# Autodesk Inventor assembly: 0008-10-02 X Axis
(part 2 of 2)
- [Insert] (2 mm): 0008-10-2018 DIN 912 - M4 x 0.7 x 40.ipt:220 ↔ 0008-10-2001 DIN 934 - M4 x 0.7.ipt:222
- [Insert]: 0008-10-2002 DIN 125 - A 4.3.ipt:225 ↔ 0008-10-2001 DIN 934 - M4 x 0.7.ipt:226
- [Insert]: 0008-10-2018 DIN 912 - M4 x 0.7 x 40.ipt:224 ↔ 0008-10-2002 DIN 125 - A 4.3.ipt:227
- [Insert] (2 mm): 0008-10-2018 DIN 912 - M4 x 0.7 x 40.ipt:224 ↔ 0008-10-2001 DIN 934 - M4 x 0.7.ipt:226
- Insert:124: 0008-10-008 X Axis suport.ipt:10 ↔ 0008-10-2002 DIN 125 - A 4.3.ipt:219
- Insert:125: 0008-10-008 X Axis suport.ipt:10 ↔ 0008-10-2002 DIN 125 - A 4.3.ipt:223
- Insert:126: 0008-10-008 X Axis suport.ipt:10 ↔ 0008-10-2002 DIN 125 - A 4.3.ipt:215
- Insert:127: 0008-10-008 X Axis suport.ipt:10 ↔ 0008-10-2002 DIN 125 - A 4.3.ipt:227
- [Insert]: 0008-10-2002 DIN 125 - A 4.3.ipt:229 ↔ 0008-10-2001 DIN 934 - M4 x 0.7.ipt:230
- [Insert]: 0008-10-2018 DIN 912 - M4 x 0.7 x 40.ipt:228 ↔ 0008-10-2002 DIN 125 - A 4.3.ipt:231
- [Insert] (2 mm): 0008-10-2018 DIN 912 - M4 x 0.7 x 40.ipt:228 ↔ 0008-10-2001 DIN 934 - M4 x 0.7.ipt:230
- [Insert]: 0008-10-2002 DIN 125 - A 4.3.ipt:233 ↔ 0008-10-2001 DIN 934 - M4 x 0.7.ipt:234
- [Insert]: 0008-10-2018 DIN 912 - M4 x 0.7 x 40.ipt:232 ↔ 0008-10-2002 DIN 125 - A 4.3.ipt:235
- [Insert] (2 mm): 0008-10-2018 DIN 912 - M4 x 0.7 x 40.ipt:232 ↔ 0008-10-2001 DIN 934 - M4 x 0.7.ipt:234
- [Insert]: 0008-10-2002 DIN 125 - A 4.3.ipt:237 ↔ 0008-10-2001 DIN 934 - M4 x 0.7.ipt:238
- [Insert]: 0008-10-2018 DIN 912 - M4 x 0.7 x 40.ipt:236 ↔ 0008-10-2002 DIN 125 - A 4.3.ipt:239
- [Insert] (2 mm): 0008-10-2018 DIN 912 - M4 x 0.7 x 40.ipt:236 ↔ 0008-10-2001 DIN 934 - M4 x 0.7.ipt:238
- [Insert]: 0008-10-2002 DIN 125 - A 4.3.ipt:241 ↔ 0008-10-2001 DIN 934 - M4 x 0.7.ipt:242
- [Insert]: 0008-10-2018 DIN 912 - M4 x 0.7 x 40.ipt:240 ↔ 0008-10-2002 DIN 125 - A 4.3.ipt:243
- [Insert] (2 mm): 0008-10-2018 DIN 912 - M4 x 0.7 x 40.ipt:240 ↔ 0008-10-2001 DIN 934 - M4 x 0.7.ipt:242
- Insert:140: 0008-10-009 X Axis suport.ipt:9 ↔ 0008-10-2002 DIN 125 - A 4.3.ipt:243
- Insert:141: 0008-10-009 X Axis suport.ipt:9 ↔ 0008-10-2002 DIN 125 - A 4.3.ipt:231
- Insert:142: 0008-10-009 X Axis suport.ipt:9 ↔ 0008-10-2002 DIN 125 - A 4.3.ipt:235
- Insert:143: 0008-10-009 X Axis suport.ipt:9 ↔ 0008-10-2002 DIN 125 - A 4.3.ipt:239
- [Insert]: 0008-10-2002 DIN 125 - A 4.3.ipt:245 ↔ 0008-10-2001 DIN 934 - M4 x 0.7.ipt:246
- [Insert]: 0008-10-2018 DIN 912 - M4 x 0.7 x 40.ipt:244 ↔ 0008-10-2002 DIN 125 - A 4.3.ipt:247
- [Insert] (2 mm): 0008-10-2018 DIN 912 - M4 x 0.7 x 40.ipt:244 ↔ 0008-10-2001 DIN 934 - M4 x 0.7.ipt:246
- [Insert]: 0008-10-2002 DIN 125 - A 4.3.ipt:249 ↔ 0008-10-2001 DIN 934 - M4 x 0.7.ipt:250
- [Insert]: 0008-10-2018 DIN 912 - M4 x 0.7 x 40.ipt:248 ↔ 0008-10-2002 DIN 125 - A 4.3.ipt:251
- [Insert] (2 mm): 0008-10-2018 DIN 912 - M4 x 0.7 x 40.ipt:248 ↔ 0008-10-2001 DIN 934 - M4 x 0.7.ipt:250
- [Insert]: 0008-10-2002 DIN 125 - A 4.3.ipt:253 ↔ 0008-10-2001 DIN 934 - M4 x 0.7.ipt:254
- [Insert]: 0008-10-2018 DIN 912 - M4 x 0.7 x 40.ipt:252 ↔ 0008-10-2002 DIN 125 - A 4.3.ipt:255
- [Insert] (2 mm): 0008-10-2018 DIN 912 - M4 x 0.7 x 40.ipt:252 ↔ 0008-10-2001 DIN 934 - M4 x 0.7.ipt:254
- [Insert]: 0008-10-2002 DIN 125 - A 4.3.ipt:257 ↔ 0008-10-2001 DIN 934 - M4 x 0.7.ipt:258
- [Insert]: 0008-10-2018 DIN 912 - M4 x 0.7 x 40.ipt:256 ↔ 0008-10-2002 DIN 125 - A 4.3.ipt:259
- [Insert] (2 mm): 0008-10-2018 DIN 912 - M4 x 0.7 x 40.ipt:256 ↔ 0008-10-2001 DIN 934 - M4 x 0.7.ipt:258
- Insert:156: 0008-10-009 X Axis suport.ipt:9 ↔ 0008-10-2002 DIN 125 - A 4.3.ipt:247
- Insert:157: 0008-10-009 X Axis suport.ipt:9 ↔ 0008-10-2002 DIN 125 - A 4.3.ipt:251
- Insert:158: 0008-10-009 X Axis suport.ipt:9 ↔ 0008-10-2002 DIN 125 - A 4.3.ipt:255
- Insert:159: 0008-10-009 X Axis suport.ipt:9 ↔ 0008-10-2002 DIN 125 - A 4.3.ipt:259
- [Insert]: 0008-10-2002 DIN 125 - A 4.3.ipt:261 ↔ 0008-10-2001 DIN 934 - M4 x 0.7.ipt:262
- [Insert]: 0008-10-2018 DIN 912 - M4 x 0.7 x 40.ipt:260 ↔ 0008-10-2002 DIN 125 - A 4.3.ipt:263
- [Insert] (2 mm): 0008-10-2018 DIN 912 - M4 x 0.7 x 40.ipt:260 ↔ 0008-10-2001 DIN 934 - M4 x 0.7.ipt:262
- [Insert]: 0008-10-2002 DIN 125 - A 4.3.ipt:265 ↔ 0008-10-2001 DIN 934 - M4 x 0.7.ipt:266
- [Insert]: 0008-10-2018 DIN 912 - M4 x 0.7 x 40.ipt:264 ↔ 0008-10-2002 DIN 125 - A 4.3.ipt:267
- [Insert] (2 mm): 0008-10-2018 DIN 912 - M4 x 0.7 x 40.ipt:264 ↔ 0008-10-2001 DIN 934 - M4 x 0.7.ipt:266
- [Insert]: 0008-10-2002 DIN 125 - A 4.3.ipt:269 ↔ 0008-10-2001 DIN 934 - M4 x 0.7.ipt:270
- [Insert]: 0008-10-2018 DIN 912 - M4 x 0.7 x 40.ipt:268 ↔ 0008-10-2002 DIN 125 - A 4.3.ipt:271
- [Insert] (2 mm): 0008-10-2018 DIN 912 - M4 x 0.7 x 40.ipt:268 ↔ 0008-10-2001 DIN 934 - M4 x 0.7.ipt:270
- Insert:172: 0008-10-009 X Axis suport.ipt:9 ↔ 0008-10-2002 DIN 125 - A 4.3.ipt:271
- Insert:173: 0008-10-009 X Axis suport.ipt:9 ↔ 0008-10-2002 DIN 125 - A 4.3.ipt:263
- Insert:174: 0008-10-009 X Axis suport.ipt:9 ↔ 0008-10-2002 DIN 125 - A 4.3.ipt:267
- Insert:175: 0008-10-2019 DIN 6912 - M4 x 50.ipt:272 ↔ 0008-10-2002 DIN 125 - A 4.3.ipt:273
- Insert:176: 0008-10-2002 DIN 125 - A 4.3.ipt:274 ↔ 0008-10-2001 DIN 934 - M4 x 0.7.ipt:275
- Insert:177 (2.7 mm): 0008-10-2019 DIN 6912 - M4 x 50.ipt:272 ↔ 0008-10-2001 DIN 934 - M4 x 0.7.ipt:275
- Insert:178: 0008-10-006 suport injectomat.ipt:1 ↔ 0008-10-2002 DIN 125 - A 4.3.ipt:273
- [Insert]: 0008-10-2019 DIN 6912 - M4 x 50.ipt:276 ↔ 0008-10-2002 DIN 125 - A 4.3.ipt:277
- [Insert]: 0008-10-2002 DIN 125 - A 4.3.ipt:278 ↔ 0008-10-2001 DIN 934 - M4 x 0.7.ipt:279
- [Insert] (2.7 mm): 0008-10-2019 DIN 6912 - M4 x 50.ipt:276 ↔ 0008-10-2001 DIN 934 - M4 x 0.7.ipt:279
- [Insert]: 0008-10-2019 DIN 6912 - M4 x 50.ipt:280 ↔ 0008-10-2002 DIN 125 - A 4.3.ipt:281
- [Insert]: 0008-10-2002 DIN 125 - A 4.3.ipt:282 ↔ 0008-10-2001 DIN 934 - M4 x 0.7.ipt:283
- [Insert] (2.7 mm): 0008-10-2019 DIN 6912 - M4 x 50.ipt:280 ↔ 0008-10-2001 DIN 934 - M4 x 0.7.ipt:283
- [Insert]: 0008-10-2019 DIN 6912 - M4 x 50.ipt:284 ↔ 0008-10-2002 DIN 125 - A 4.3.ipt:285
- [Insert]: 0008-10-2002 DIN 125 - A 4.3.ipt:286 ↔ 0008-10-2001 DIN 934 - M4 x 0.7.ipt:287
- [Insert] (2.7 mm): 0008-10-2019 DIN 6912 - M4 x 50.ipt:284 ↔ 0008-10-2001 DIN 934 - M4 x 0.7.ipt:287
- [Insert]: 0008-10-2019 DIN 6912 - M4 x 50.ipt:288 ↔ 0008-10-2002 DIN 125 - A 4.3.ipt:289
- [Insert]: 0008-10-2002 DIN 125 - A 4.3.ipt:290 ↔ 0008-10-2001 DIN 934 - M4 x 0.7.ipt:291
- [Insert] (2.7 mm): 0008-10-2019 DIN 6912 - M4 x 50.ipt:288 ↔ 0008-10-2001 DIN 934 - M4 x 0.7.ipt:291
- [Insert]: 0008-10-2019 DIN 6912 - M4 x 50.ipt:292 ↔ 0008-10-2002 DIN 125 - A 4.3.ipt:293
- [Insert]: 0008-10-2002 DIN 125 - A 4.3.ipt:294 ↔ 0008-10-2001 DIN 934 - M4 x 0.7.ipt:295
- [Insert] (2.7 mm): 0008-10-2019 DIN 6912 - M4 x 50.ipt:292 ↔ 0008-10-2001 DIN 934 - M4 x 0.7.ipt:295
- [Insert]: 0008-10-2019 DIN 6912 - M4 x 50.ipt:296 ↔ 0008-10-2002 DIN 125 - A 4.3.ipt:297
- [Insert]: 0008-10-2002 DIN 125 - A 4.3.ipt:298 ↔ 0008-10-2001 DIN 934 - M4 x 0.7.ipt:299
- [Insert] (2.7 mm): 0008-10-2019 DIN 6912 - M4 x 50.ipt:296 ↔ 0008-10-2001 DIN 934 - M4 x 0.7.ipt:299
- Insert:197: 0008-10-006 suport injectomat.ipt:1 ↔ 0008-10-2002 DIN 125 - A 4.3.ipt:277
- Insert:198: 0008-10-006 suport injectomat.ipt:1 ↔ 0008-10-2002 DIN 125 - A 4.3.ipt:285
- Insert:199: 0008-10-006 suport injectomat.ipt:1 ↔ 0008-10-2002 DIN 125 - A 4.3.ipt:281
- Insert:200: 0008-10-006 suport injectomat.ipt:1 ↔ 0008-10-2002 DIN 125 - A 4.3.ipt:289
- Insert:201: 0008-10-006 suport injectomat.ipt:1 ↔ 0008-10-2002 DIN 125 - A 4.3.ipt:293
- Insert:202: 0008-10-006 suport injectomat.ipt:1 ↔ 0008-10-2002 DIN 125 - A 4.3.ipt:297
- [Insert]: 0008-10-2019 DIN 6912 - M4 x 50.ipt:300 ↔ 0008-10-2002 DIN 125 - A 4.3.ipt:301
- [Insert]: 0008-10-2002 DIN 125 - A 4.3.ipt:302 ↔ 0008-10-2001 DIN 934 - M4 x 0.7.ipt:303
- [Insert] (2.7 mm): 0008-10-2019 DIN 6912 - M4 x 50.ipt:300 ↔ 0008-10-2001 DIN 934 - M4 x 0.7.ipt:303
- [Insert]: 0008-10-2019 DIN 6912 - M4 x 50.ipt:304 ↔ 0008-10-2002 DIN 125 - A 4.3.ipt:305
- [Insert]: 0008-10-2002 DIN 125 - A 4.3.ipt:306 ↔ 0008-10-2001 DIN 934 - M4 x 0.7.ipt:307
- [Insert] (2.7 mm): 0008-10-2019 DIN 6912 - M4 x 50.ipt:304 ↔ 0008-10-2001 DIN 934 - M4 x 0.7.ipt:307
- [Insert]: 0008-10-2019 DIN 6912 - M4 x 50.ipt:308 ↔ 0008-10-2002 DIN 125 - A 4.3.ipt:309
- [Insert]: 0008-10-2002 DIN 125 - A 4.3.ipt:310 ↔ 0008-10-2001 DIN 934 - M4 x 0.7.ipt:311
- [Insert] (2.7 mm): 0008-10-2019 DIN 6912 - M4 x 50.ipt:308 ↔ 0008-10-2001 DIN 934 - M4 x 0.7.ipt:311
- Insert:212: 0008-10-006 suport injectomat.ipt:1 ↔ 0008-10-2002 DIN 125 - A 4.3.ipt:305
- Insert:213: 0008-10-006 suport injectomat.ipt:1 ↔ 0008-10-2002 DIN 125 - A 4.3.ipt:301
- Insert:214: 0008-10-006 suport injectomat.ipt:1 ↔ 0008-10-2002 DIN 125 - A 4.3.ipt:309
- Insert:215: 0008-10-2003DIN 6912 - M4 x 35.ipt:312 ↔ 0008-10-2002 DIN 125 - A 4.3.ipt:313
- Insert:216: 0008-10-2002 DIN 125 - A 4.3.ipt:314 ↔ 0008-10-2001 DIN 934 - M4 x 0.7.ipt:315
- Insert:217 (4.8 mm): 0008-10-2003DIN 6912 - M4 x 35.ipt:312 ↔ 0008-10-2001 DIN 934 - M4 x 0.7.ipt:315
- Insert:218: 0008-10-013 Supăort Piulita Axa Z.ipt:22 ↔ 0008-10-2002 DIN 125 - A 4.3.ipt:313
- [Insert]: 0008-10-2003DIN 6912 - M4 x 35.ipt:44 ↔ 0008-10-2002 DIN 125 - A 4.3.ipt:45
- [Insert]: 0008-10-2002 DIN 125 - A 4.3.ipt:46 ↔ 0008-10-2001 DIN 934 - M4 x 0.7.ipt:47
- [Insert] (4.8 mm): 0008-10-2003DIN 6912 - M4 x 35.ipt:44 ↔ 0008-10-2001 DIN 934 - M4 x 0.7.ipt:47
- [Insert]: 0008-10-2003DIN 6912 - M4 x 35.ipt:48 ↔ 0008-10-2002 DIN 125 - A 4.3.ipt:49
- [Insert]: 0008-10-2002 DIN 125 - A 4.3.ipt:50 ↔ 0008-10-2001 DIN 934 - M4 x 0.7.ipt:51
- [Insert] (4.8 mm): 0008-10-2003DIN 6912 - M4 x 35.ipt:48 ↔ 0008-10-2001 DIN 934 - M4 x 0.7.ipt:51
- [Insert]: 0008-10-2003DIN 6912 - M4 x 35.ipt:52 ↔ 0008-10-2002 DIN 125 - A 4.3.ipt:53
- [Insert]: 0008-10-2002 DIN 125 - A 4.3.ipt:54 ↔ 0008-10-2001 DIN 934 - M4 x 0.7.ipt:55
- [Insert] (4.8 mm): 0008-10-2003DIN 6912 - M4 x 35.ipt:52 ↔ 0008-10-2001 DIN 934 - M4 x 0.7.ipt:55
- Insert:228: 0008-10-013 Supăort Piulita Axa Z.ipt:22 ↔ 0008-10-2002 DIN 125 - A 4.3.ipt:53
- Insert:229: 0008-10-013 Supăort Piulita Axa Z.ipt:22 ↔ 0008-10-2002 DIN 125 - A 4.3.ipt:49
- Insert:230: 0008-10-013 Supăort Piulita Axa Z.ipt:22 ↔ 0008-10-2002 DIN 125 - A 4.3.ipt:45
- [Insert]: 0008-10-2003DIN 6912 - M4 x 35.ipt:56 ↔ 0008-10-2002 DIN 125 - A 4.3.ipt:57
- [Insert]: 0008-10-2002 DIN 125 - A 4.3.ipt:58 ↔ 0008-10-2001 DIN 934 - M4 x 0.7.ipt:59
- [Insert]: 0008-10-2003DIN 6912 - M4 x 35.ipt:56 ↔ 0008-10-2001 DIN 934 - M4 x 0.7.ipt:59
- Insert:234: 0008-10-007 Contra suport injectomat.ipt:6 ↔ 0008-10-2002 DIN 125 - A 4.3.ipt:57
- [Insert]: 0008-10-2003DIN 6912 - M4 x 35.ipt:60 ↔ 0008-10-2002 DIN 125 - A 4.3.ipt:61
- [Insert]: 0008-10-2002 DIN 125 - A 4.3.ipt:62 ↔ 0008-10-2001 DIN 934 - M4 x 0.7.ipt:63
- [Insert]: 0008-10-2003DIN 6912 - M4 x 35.ipt:60 ↔ 0008-10-2001 DIN 934 - M4 x 0.7.ipt:63
- Insert:238: 0008-10-007 Contra suport injectomat.ipt:6 ↔ 0008-10-2002 DIN 125 - A 4.3.ipt:61
- [Insert]: 0008-10-2003DIN 6912 - M4 x 35.ipt:64 ↔ 0008-10-2002 DIN 125 - A 4.3.ipt:65
- [Insert]: 0008-10-2002 DIN 125 - A 4.3.ipt:66 ↔ 0008-10-2001 DIN 934 - M4 x 0.7.ipt:67
- [Insert] (4.8 mm): 0008-10-2003DIN 6912 - M4 x 35.ipt:64 ↔ 0008-10-2001 DIN 934 - M4 x 0.7.ipt:67
- [Insert]: 0008-10-2003DIN 6912 - M4 x 35.ipt:68 ↔ 0008-10-2002 DIN 125 - A 4.3.ipt:69
- [Insert]: 0008-10-2002 DIN 125 - A 4.3.ipt:70 ↔ 0008-10-2001 DIN 934 - M4 x 0.7.ipt:71
- [Insert] (4.8 mm): 0008-10-2003DIN 6912 - M4 x 35.ipt:68 ↔ 0008-10-2001 DIN 934 - M4 x 0.7.ipt:71
- [Insert]: 0008-10-2003DIN 6912 - M4 x 35.ipt:72 ↔ 0008-10-2002 DIN 125 - A 4.3.ipt:73
- [Insert]: 0008-10-2002 DIN 125 - A 4.3.ipt:74 ↔ 0008-10-2001 DIN 934 - M4 x 0.7.ipt:75
- [Insert] (4.8 mm): 0008-10-2003DIN 6912 - M4 x 35.ipt:72 ↔ 0008-10-2001 DIN 934 - M4 x 0.7.ipt:75
- [Insert]: 0008-10-2003DIN 6912 - M4 x 35.ipt:76 ↔ 0008-10-2002 DIN 125 - A 4.3.ipt:77
- [Insert]: 0008-10-2002 DIN 125 - A 4.3.ipt:78 ↔ 0008-10-2001 DIN 934 - M4 x 0.7.ipt:79
- [Insert] (4.8 mm): 0008-10-2003DIN 6912 - M4 x 35.ipt:76 ↔ 0008-10-2001 DIN 934 - M4 x 0.7.ipt:79
- Insert:251: 0008-10-013 Supăort Piulita Axa Z.ipt:24 ↔ 0008-10-2002 DIN 125 - A 4.3.ipt:77
- Insert:252: 0008-10-013 Supăort Piulita Axa Z.ipt:24 ↔ 0008-10-2002 DIN 125 - A 4.3.ipt:73
- Insert:253: 0008-10-013 Supăort Piulita Axa Z.ipt:24 ↔ 0008-10-2002 DIN 125 - A 4.3.ipt:65
- Insert:254: 0008-10-013 Supăort Piulita Axa Z.ipt:24 ↔ 0008-10-2002 DIN 125 - A 4.3.ipt:69
- [Insert]: 0008-10-2006 DIN 7984 - M3 x 16.ipt:80 ↔ 0008-10-2009 DIN 555-5 - M3.ipt:81
- Insert:256: 0008-10-1004 Piulita.ipt:23 ↔ 0008-10-2006 DIN 7984 - M3 x 16.ipt:80
- [Insert]: 0008-10-2006 DIN 7984 - M3 x 16.ipt:82 ↔ 0008-10-2009 DIN 555-5 - M3.ipt:83
- [Insert]: 0008-10-2006 DIN 7984 - M3 x 16.ipt:84 ↔ 0008-10-2009 DIN 555-5 - M3.ipt:85
- [Insert]: 0008-10-2006 DIN 7984 - M3 x 16.ipt:86 ↔ 0008-10-2009 DIN 555-5 - M3.ipt:87
- Insert:260: 0008-10-1004 Piulita.ipt:23 ↔ 0008-10-2006 DIN 7984 - M3 x 16.ipt:84
- Insert:261: 0008-10-1004 Piulita.ipt:23 ↔ 0008-10-2006 DIN 7984 - M3 x 16.ipt:82
- Insert:262: 0008-10-1004 Piulita.ipt:23 ↔ 0008-10-2006 DIN 7984 - M3 x 16.ipt:86
- [Insert]: 0008-10-2006 DIN 7984 - M3 x 16.ipt:88 ↔ 0008-10-2009 DIN 555-5 - M3.ipt:89
- [Insert]: 0008-10-2006 DIN 7984 - M3 x 16.ipt:90 ↔ 0008-10-2009 DIN 555-5 - M3.ipt:91
- [Insert]: 0008-10-2006 DIN 7984 - M3 x 16.ipt:92 ↔ 0008-10-2009 DIN 555-5 - M3.ipt:93
- [Insert]: 0008-10-2006 DIN 7984 - M3 x 16.ipt:94 ↔ 0008-10-2009 DIN 555-5 - M3.ipt:95
- Insert:267: 0008-10-1004 Piulita.ipt:25 ↔ 0008-10-2006 DIN 7984 - M3 x 16.ipt:94
- Insert:268: 0008-10-1004 Piulita.ipt:25 ↔ 0008-10-2006 DIN 7984 - M3 x 16.ipt:88
- Insert:269: 0008-10-1004 Piulita.ipt:25 ↔ 0008-10-2006 DIN 7984 - M3 x 16.ipt:90
- Insert:270: 0008-10-1004 Piulita.ipt:25 ↔ 0008-10-2006 DIN 7984 - M3 x 16.ipt:92
- [Insert]: 0008-10-2009 DIN 555-5 - M3.ipt:99 ↔ 0008-10-2005 DIN 125 - A 3.2.ipt:100
- Insert:274: 0008-10-2020 DIN 7991 - M3  x  16.ipt:98 ↔ 0008-10-2009 DIN 555-5 - M3.ipt:99
- [Insert]: 0008-10-2009 DIN 555-5 - M3.ipt:102 ↔ 0008-10-2005 DIN 125 - A 3.2.ipt:103
- [Insert]: 0008-10-2020 DIN 7991 - M3  x  16.ipt:101 ↔ 0008-10-2009 DIN 555-5 - M3.ipt:102
- [Insert]: 0008-10-2009 DIN 555-5 - M3.ipt:105 ↔ 0008-10-2005 DIN 125 - A 3.2.ipt:106
- [Insert]: 0008-10-2020 DIN 7991 - M3  x  16.ipt:104 ↔ 0008-10-2009 DIN 555-5 - M3.ipt:105
- [Insert]: 0008-10-2009 DIN 555-5 - M3.ipt:108 ↔ 0008-10-2005 DIN 125 - A 3.2.ipt:109
- [Insert]: 0008-10-2020 DIN 7991 - M3  x  16.ipt:107 ↔ 0008-10-2009 DIN 555-5 - M3.ipt:108
- Insert:283 (2 mm): 0008-10-046 Fixare axa si port cablu.ipt:21 ↔ 0008-10-2020 DIN 7991 - M3  x  16.ipt:104
- Insert:284 (-2 mm): 0008-10-046 Fixare axa si port cablu.ipt:21 ↔ 0008-10-2020 DIN 7991 - M3  x  16.ipt:107
- Insert:285: 0008-10-2004 DIN 7984 - M3 x 20.ipt:110 ↔ 0008-10-2005 DIN 125 - A 3.2.ipt:111
- [Insert]: 0008-10-2004 DIN 7984 - M3 x 20.ipt:112 ↔ 0008-10-2005 DIN 125 - A 3.2.ipt:113
- [Insert]: 0008-10-2004 DIN 7984 - M3 x 20.ipt:114 ↔ 0008-10-2005 DIN 125 - A 3.2.ipt:115
- [Insert]: 0008-10-2004 DIN 7984 - M3 x 20.ipt:116 ↔ 0008-10-2005 DIN 125 - A 3.2.ipt:117
- Insert:289: 0008-10-009 X Axis suport.ipt:9 ↔ 0008-10-2005 DIN 125 - A 3.2.ipt:117
- Insert:290: 0008-10-009 X Axis suport.ipt:9 ↔ 0008-10-2005 DIN 125 - A 3.2.ipt:115
- Insert:291: 0008-10-009 X Axis suport.ipt:9 ↔ 0008-10-2005 DIN 125 - A 3.2.ipt:113
- Insert:292: 0008-10-009 X Axis suport.ipt:9 ↔ 0008-10-2005 DIN 125 - A 3.2.ipt:111
- Insert:293: 0008-10-012 Intinzator X.ipt:15 ↔ 0008-10-2021 DIN 7984 - M5 x 30.ipt:118
- Insert:294: 0008-10-012 Intinzator X.ipt:15 ↔ 0008-10-2012 DIN 125 - A 5.3.ipt:119
- Insert:295: 0008-10-2022 DIN 934 - M5 x 0.8.ipt:35 ↔ 0008-10-2012 DIN 125 - A 5.3.ipt:119
- [Insert]: 0008-10-2002 DIN 125 - A 4.3.ipt:37 ↔ 0008-10-2001 DIN 934 - M4 x 0.7.ipt:38
- [Insert]: 0008-10-2018 DIN 912 - M4 x 0.7 x 40.ipt:36 ↔ 0008-10-2002 DIN 125 - A 4.3.ipt:39
- [Insert] (2 mm): 0008-10-2018 DIN 912 - M4 x 0.7 x 40.ipt:36 ↔ 0008-10-2001 DIN 934 - M4 x 0.7.ipt:38
- [Insert]: 0008-10-2002 DIN 125 - A 4.3.ipt:41 ↔ 0008-10-2001 DIN 934 - M4 x 0.7.ipt:42
- [Insert]: 0008-10-2018 DIN 912 - M4 x 0.7 x 40.ipt:40 ↔ 0008-10-2002 DIN 125 - A 4.3.ipt:43
- [Insert] (2 mm): 0008-10-2018 DIN 912 - M4 x 0.7 x 40.ipt:40 ↔ 0008-10-2001 DIN 934 - M4 x 0.7.ipt:42
- Insert:302: 0008-10-008 X Axis suport.ipt:10 ↔ 0008-10-2002 DIN 125 - A 4.3.ipt:39
- Insert:303: 0008-10-008 X Axis suport.ipt:10 ↔ 0008-10-2002 DIN 125 - A 4.3.ipt:43
- Mate:197: 0008-10-008 X Axis suport.ipt:10 ↔ 0008-10-1023 Compress Spring11.ipt:316
- Mate:198: 0008-10-2018 DIN 912 - M4 x 0.7 x 40.ipt:36 ↔ 0008-10-1023 Compress Spring11.ipt:316
- [Insert]: 0008-10-2009 DIN 555-5 - M3.ipt:319 ↔ 0008-10-2005 DIN 125 - A 3.2.ipt:320
- [Insert]: 0008-10-2020 DIN 7991 - M3  x  16.ipt:318 ↔ 0008-10-2009 DIN 555-5 - M3.ipt:319
- [Insert]: 0008-10-2009 DIN 555-5 - M3.ipt:322 ↔ 0008-10-2005 DIN 125 - A 3.2.ipt:323
- [Insert]: 0008-10-2020 DIN 7991 - M3  x  16.ipt:321 ↔ 0008-10-2009 DIN 555-5 - M3.ipt:322
- Insert:308 (-2 mm): 0008-10-046 Fixare axa si port cablu.ipt:21 ↔ 0008-10-2020 DIN 7991 - M3  x  16.ipt:321
- Insert:309 (-2 mm): 0008-10-046 Fixare axa si port cablu.ipt:21 ↔ 0008-10-2020 DIN 7991 - M3  x  16.ipt:318
- Mate:199: 0008-10-007 Contra suport injectomat.ipt:6 ↔ 0008-20-1003 Switch.ipt:28
- Flush:130: 0008-10-007 Contra suport injectomat.ipt:6 ↔ 0008-20-1003 Switch.ipt:28
- Insert:310: 0008-20-1003 Switch.ipt:28 ↔ 0008-10-2006 DIN 7984 - M3 x 16.ipt:96
- Insert:311: 0008-20-1003 Switch.ipt:28 ↔ 0008-10-2006 DIN 7984 - M3 x 16.ipt:97
- Insert:312 (-2 mm): 0008-10-007 Contra suport injectomat.ipt:6 ↔ 0008-10-2020 DIN 7991 - M3  x  16.ipt:98
- Insert:313 (-2 mm): 0008-10-007 Contra suport injectomat.ipt:6 ↔ 0008-10-2020 DIN 7991 - M3  x  16.ipt:101
- Mate:200: 0008-10-046 Fixare axa si port cablu.ipt:21 ↔ 0008-10-1025 Wire chain.ipt:325
- Flush:131: 0008-10-046 Fixare axa si port cablu.ipt:21 ↔ 0008-10-1025 Wire chain.ipt:325
- Flush:132: 0008-10-046 Fixare axa si port cablu.ipt:21 ↔ 0008-10-1025 Wire chain.ipt:325
- Mate:201: 0008-10-1004 Piulita.ipt:25 ↔ 0008-10-04 Z axis_Shrinkwrap.ipt:326
- Mate:202: 0008-10-1013 LMK 10 Bearing.ipt:18 ↔ 0008-10-04 Z axis_Shrinkwrap.ipt:326
## Named parameters: d479_d475 = 0 mm, d480_d477 = 0 mm, d481_d478 = 3.8 mm, d483_d475 = 0 mm, d484_d477 = 0 mm, d485_d478 = 3.8 mm, d486_d475 = 0 mm, d487_d477 = 0 mm, d488_d478 = 3.8 mm, d491_d475 = 0 mm, d492_d477 = 0 mm, d493_d478 = 3.8 mm, d494_d475 = 0 mm, d495_d477 = 0 mm, d496_d478 = 3.8 mm, d497_d475 = 0 mm, d498_d477 = 0 mm, d499_d478 = 3.8 mm, d500_d475 = 0 mm, d501_d477 = 0 mm, d502_d478 = 3.8 mm, d507_d475 = 0 mm, d508_d477 = 0 mm, d509_d478 = 3.8 mm, d510_d475 = 0 mm, d511_d477 = 0 mm, d512_d478 = 3.8 mm, d513_d475 = 0 mm, d514_d477 = 0 mm, d515_d478 = 3.8 mm, d516_d475 = 0 mm, d517_d477 = 0 mm, d518_d478 = 3.8 mm, d523_d475 = 0 mm, d524_d477 = 0 mm, d525_d478 = 3.8 mm, d526_d475 = 0 mm, d527_d477 = 0 mm, d528_d478 = 3.8 mm, d529_d475 = 0 mm, d530_d477 = 0 mm, d531_d478 = 3.8 mm, d532_d475 = 0 mm, d533_d477 = 0 mm, d534_d478 = 3.8 mm, d539_d533_d477 = 0 mm, d543_d539_d533_d477 = 0 mm, d544_d540 = 0 mm, d545_d541 = 2 mm, d547_d539_d533_d477 = 0 mm, d548_d540 = 0 mm, d549_d541 = 2 mm, d550_d539_d533_d477 = 0 mm, d551_d540 = 0 mm, d552_d541 = 2 mm, d555_d539_d533_d477 = 0 mm, d556_d540 = 0 mm, d557_d541 = 2 mm, d558_d539_d533_d477 = 0 mm, d559_d540 = 0 mm, d560_d541 = 2 mm, d561_d539_d533_d477 = 0 mm, d562_d540 = 0 mm, d563_d541 = 2 mm, d567_d539_d533_d477 = 0 mm, d568_d540 = 0 mm, d569_d541 = 2 mm, d570_d539_d533_d477 = 0 mm, d571_d540 = 0 mm, d572_d541 = 2 mm, d573_d539_d533_d477 = 0 mm, d574_d540 = 0 mm, d575_d541 = 2 mm, d576_d539_d533_d477 = 0 mm, d577_d540 = 0 mm, d578_d541 = 2 mm, d583_d539_d533_d477 = 0 mm, d584_d540 = 0 mm, d585_d541 = 2 mm, d586_d539_d533_d477 = 0 mm, d587_d540 = 0 mm, d588_d541 = 2 mm, d589_d539_d533_d477 = 0 mm, d590_d540 = 0 mm, d591_d541 = 2 mm, d592_d539_d533_d477 = 0 mm, d593_d540 = 0 mm, d594_d541 = 2 mm, d599_d539_d533_d477 = 0 mm, d600_d540 = 0 mm, d601_d541 = 2 mm, d602_d539_d533_d477 = 0 mm, d603_d540 = 0 mm, d604_d541 = 2 mm, d605_d539_d533_d477 = 0 mm, d606_d540 = 0 mm, d607_d541 = 2 mm, d608_d539_d533_d477 = 0 mm, d609_d540 = 0 mm, d610_d541 = 2 mm, d615_d539_d533_d477 = 0 mm, d616_d540 = 0 mm, d617_d541 = 2 mm, d618_d539_d533_d477 = 0 mm, d619_d540 = 0 mm, d620_d541 = 2 mm, d624_d539_d533_d477 = 0 mm, d625_d540 = 0 mm, d626_d541 = 2 mm, d634_d630 = 0 mm, d635_d631 = 0 mm, d636_d632 = 2.7 mm, d637_d630 = 0 mm, d638_d631 = 0 mm, d639_d632 = 2.7 mm, d640_d630 = 0 mm, d641_d631 = 0 mm, d642_d632 = 2.7 mm, d643_d630 = 0 mm, d644_d631 = 0 mm, d645_d632 = 2.7 mm, d646_d630 = 0 mm, d647_d631 = 0 mm, d648_d632 = 2.7 mm, d649_d630 = 0 mm, d650_d631 = 0 mm, d651_d632 = 2.7 mm, d658_d630 = 0 mm, d659_d631 = 0 mm, d660_d632 = 2.7 mm, d661_d630 = 0 mm, d662_d631 = 0 mm, d663_d632 = 2.7 mm, d664_d630 = 0 mm, d665_d631 = 0 mm, d666_d632 = 2.7 mm, d674_d670 = 0 mm, d675_d671 = 0 mm, d676_d672 = 4.8 mm, d677_d670 = 0 mm, d678_d671 = 0 mm, d679_d672 = 4.8 mm, d680_d670 = 0 mm, d681_d671 = 0 mm, d682_d672 = 4.8 mm, d686_d670 = 0 mm, d687_d671 = 0 mm, d688_d672 = 0 mm, d690_d686_d670 = 0 mm, d691_d687_d671 = 0 mm, d692_d688_d672 = 0 mm, d694_d677_d670 = 0 mm, d695_d678_d671 = 0 mm, d696_d679_d672 = 4.8 mm, d697_d677_d670 = 0 mm, d698_d678_d671 = 0 mm, d699_d679_d672 = 4.8 mm, d700_d677_d670 = 0 mm, d701_d678_d671 = 0 mm, d702_d679_d672 = 4.8 mm, d703_d677_d670 = 0 mm, d704_d678_d671 = 0 mm, d705_d679_d672 = 4.8 mm, d712_d66 = 0 mm, d713_d66 = 0 mm, d714_d66 = 0 mm, d718_d66 = 0 mm, d719_d66 = 0 mm, d720_d66 = 0 mm, d721_d66 = 0 mm, d735_d2 = 0 mm, d736_d732 = 0 mm, d738_d2 = 0 mm, d739_d732 = 0 mm, d740_d2 = 0 mm, d741_d732 = 0 mm, d745_d744 = 0 mm, d746_d744 = 0 mm, d747_d744 = 0 mm, d755_d558_d539_d533_d477 = 0 mm, d756_d559_d540 = 0 mm, d757_d560_d541 = 2 mm, d758_d558_d539_d533_d477 = 0 mm, d759_d559_d540 = 0 mm, d760_d560_d541 = 2 mm, d769_d738_d2 = 0 mm, d770_d739_d732 = 0 mm, d771_d738_d2 = 0 mm, d772_d739_d732 = 0 mm
